# Autodesk Inventor assembly: _MK-1_Assembly
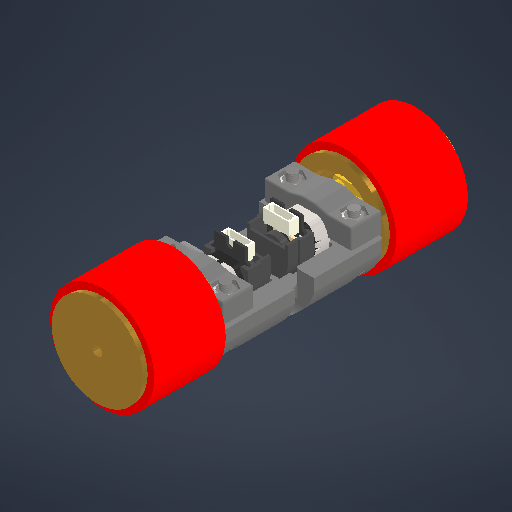
[picture p0: Inventor's stored thumbnail of the model, 512x512]
Saved by Autodesk Inventor 2027 (Build 310192000, 192)
## iProperties
Created: 2026-04-22
Part Number: _MK-1_Assembly
Document SubType Name: Assembly
Designer: Vadim
Author: Vadim
## Documents named in this file (12)
- C:\Users\Vadim\GitHub\NeoSumec\NeoSumec-MiniSumo-MECH\_MK-1_\_MK-1_Assembly.iam
- C:\Users\Vadim\GitHub\NeoSumec\NeoSumec-MiniSumo-MECH\_MK-1_\Models\3D_Print\MotorMountBottom.ipt
- C:\Users\Vadim\GitHub\NeoSumec\NeoSumec-MiniSumo-MECH\_MK-1_\Models\3D_Print\MotorClamp.ipt
- C:\Users\Vadim\GitHub\NeoSumec\NeoSumec-MiniSumo-MECH\_MK-1_\Models\Metal\pipe.ipt
- C:\Users\Vadim\GitHub\NeoSumec\NeoSumec-MiniSumo-MECH\_MK-1_\Models\Metal\Wheel.ipt
- C:\Users\Vadim\GitHub\NeoSumec\NeoSumec-MiniSumo-MECH\_MK-1_\Models\3rd-party_comp\Pololu Micro Metal Gearmotor 3D (STEP) Models\With Encoder, Side Connector\mmgm-cb-enc-side-con\mmgm-cb-enc-side-con\mmgm-cb-enc-side-con.ipt
- C:\Users\Vadim\GitHub\NeoSumec\NeoSumec-MiniSumo-MECH\_MK-1_\Models\Other technology\silicon bublebum.ipt
- C:\Users\Vadim\GitHub\NeoSumec\NeoSumec-MiniSumo-MECH\_MK-1_\SpojMat\DIN 934 - M3 x 0,5.ipt
- C:\Users\Vadim\GitHub\NeoSumec\NeoSumec-MiniSumo-MECH\_MK-1_\SpojMat\ISO 14580 M3x25-4.8.ipt
- C:\Users\Vadim\GitHub\NeoSumec\NeoSumec-MiniSumo-MECH\_MK-1_\SpojMat\ISO 14581 - M3x16-4.8.ipt
- C:\Users\Vadim\GitHub\NeoSumec\NeoSumec-MiniSumo-MECH\_MK-1_\SpojMat\ISO 14581 - M3x20-4.8.ipt
- C:\Users\Vadim\GitHub\NeoSumec\NeoSumec-MiniSumo-MECH\_MK-1_\SpojMat\DIN 916 - M3  x  6.ipt
## Components (23 placed, 11 different names)
1. MotorMountBottom:1 — Proti sobě:1, Proti sobě:2, Proti sobě:3, Proti sobě:4, Proti sobě:7, Proti sobě:10, Proti sobě:15, Stejný směr:1, Proti sobě:17, Proti sobě:19, Proti sobě:21, Proti sobě:34, Proti sobě:35, Proti sobě:36, Proti sobě:37, Proti sobě:38, Proti sobě:39, Proti sobě:40, Proti sobě:41
2. MotorClamp:1 — Proti sobě:18, Proti sobě:19, Proti sobě:24, Proti sobě:25, Proti sobě:26, Proti sobě:27, Proti sobě:32, Proti sobě:33
3. MotorClamp:2 — Proti sobě:16, Proti sobě:17, Proti sobě:22, Proti sobě:23, Proti sobě:28, Proti sobě:29, Proti sobě:30, Proti sobě:31
4. pipe:1 — Proti sobě:15, Stejný směr:1, Proti sobě:20
5. Wheel:1 — Proti sobě:5, Proti sobě:6, Proti sobě:7, Proti sobě:11, Proti sobě:14, Proti sobě:42, Proti sobě:44
6. Wheel:2 — Proti sobě:8, Proti sobě:9, Proti sobě:10, Proti sobě:12, Proti sobě:13, Proti sobě:45, Proti sobě:46
7. silicon bublebum:1 — Proti sobě:11, Proti sobě:14
8. silicon bublebum:2 — Proti sobě:12, Proti sobě:13
9. mmgm-cb-enc-side-con:1 — Proti sobě:1, Proti sobě:2, Proti sobě:5, Proti sobě:6, Proti sobě:18, Proti sobě:43, Proti sobě:49
10. mmgm-cb-enc-side-con:2 — Proti sobě:3, Proti sobě:4, Proti sobě:8, Proti sobě:9, Proti sobě:16, Proti sobě:47, Proti sobě:48
11. ISO 14580 M3x25-4.8:1 — Proti sobě:20, Proti sobě:21
12. DIN 916 - M3  x  6:1 — Proti sobě:42, Proti sobě:43
13. DIN 916 - M3  x  6:2 — Proti sobě:44, Proti sobě:49
14. DIN 916 - M3  x  6:3 — Proti sobě:45, Proti sobě:47
15. DIN 916 - M3  x  6:4 — Proti sobě:46, Proti sobě:48
16. ISO 14581 - M3x16-4.8:1 — Proti sobě:36, Proti sobě:37
17. ISO 14581 - M3x16-4.8:2 — Proti sobě:38, Proti sobě:39
18. ISO 14581 - M3x20-4.8:1 — Proti sobě:34, Proti sobě:35
19. ISO 14581 - M3x20-4.8:2 — Proti sobě:40, Proti sobě:41
20. DIN 934 - M3 x 0,5:1 — Proti sobě:25, Proti sobě:26, Proti sobě:33
21. DIN 934 - M3 x 0,5:2 — Proti sobě:24, Proti sobě:27, Proti sobě:32
22. DIN 934 - M3 x 0,5:3 — Proti sobě:22, Proti sobě:29, Proti sobě:30
23. DIN 934 - M3 x 0,5:4 — Proti sobě:23, Proti sobě:28, Proti sobě:31
## Relationships (50: Mate 49, Flush 1)
- Proti sobě:1 [Mate]: MotorMountBottom:1 ↔ mmgm-cb-enc-side-con:1
- Proti sobě:2 [Mate] (0.125 mm): MotorMountBottom:1 ↔ mmgm-cb-enc-side-con:1
- Proti sobě:3 [Mate]: MotorMountBottom:1 ↔ mmgm-cb-enc-side-con:2
- Proti sobě:4 [Mate] (0.125 mm): MotorMountBottom:1 ↔ mmgm-cb-enc-side-con:2
- Proti sobě:5 [Mate]: Wheel:1 ↔ mmgm-cb-enc-side-con:1
- Proti sobě:6 [Mate] (0.1 mm): Wheel:1 ↔ mmgm-cb-enc-side-con:1
- Proti sobě:7 [Mate] (0.25 mm): MotorMountBottom:1 ↔ Wheel:1
- Proti sobě:8 [Mate]: Wheel:2 ↔ mmgm-cb-enc-side-con:2
- Proti sobě:9 [Mate] (0.15 mm): Wheel:2 ↔ mmgm-cb-enc-side-con:2
- Proti sobě:10 [Mate] (0.25 mm): MotorMountBottom:1 ↔ Wheel:2
- Proti sobě:11 [Mate]: Wheel:1 ↔ silicon bublebum:1
- Proti sobě:12 [Mate]: Wheel:2 ↔ silicon bublebum:2
- Proti sobě:13 [Mate]: Wheel:2 ↔ silicon bublebum:2
- Proti sobě:14 [Mate]: Wheel:1 ↔ silicon bublebum:1
- Proti sobě:15 [Mate]: MotorMountBottom:1 ↔ pipe:1
- Stejný směr:1 [Flush]: MotorMountBottom:1 ↔ pipe:1
- Proti sobě:16 [Mate]: MotorClamp:2 ↔ mmgm-cb-enc-side-con:2
- Proti sobě:17 [Mate]: MotorMountBottom:1 ↔ MotorClamp:2
- Proti sobě:18 [Mate]: MotorClamp:1 ↔ mmgm-cb-enc-side-con:1
- Proti sobě:19 [Mate]: MotorMountBottom:1 ↔ MotorClamp:1
- Proti sobě:20 [Mate]: pipe:1 ↔ ISO 14580 M3x25-4.8:1
- Proti sobě:21 [Mate]: MotorMountBottom:1 ↔ ISO 14580 M3x25-4.8:1
- Proti sobě:22 [Mate]: MotorClamp:2 ↔ DIN 934 - M3 x 0,5:3
- Proti sobě:23 [Mate]: MotorClamp:2 ↔ DIN 934 - M3 x 0,5:4
- Proti sobě:24 [Mate]: MotorClamp:1 ↔ DIN 934 - M3 x 0,5:2
- Proti sobě:25 [Mate]: MotorClamp:1 ↔ DIN 934 - M3 x 0,5:1
- Proti sobě:26 [Mate] (0.1 mm): MotorClamp:1 ↔ DIN 934 - M3 x 0,5:1
- Proti sobě:27 [Mate] (0.1 mm): MotorClamp:1 ↔ DIN 934 - M3 x 0,5:2
- Proti sobě:28 [Mate] (0.1 mm): MotorClamp:2 ↔ DIN 934 - M3 x 0,5:4
- Proti sobě:29 [Mate] (0.1 mm): MotorClamp:2 ↔ DIN 934 - M3 x 0,5:3
- Proti sobě:30 [Mate]: MotorClamp:2 ↔ DIN 934 - M3 x 0,5:3
- Proti sobě:31 [Mate]: MotorClamp:2 ↔ DIN 934 - M3 x 0,5:4
- Proti sobě:32 [Mate]: MotorClamp:1 ↔ DIN 934 - M3 x 0,5:2
- Proti sobě:33 [Mate]: MotorClamp:1 ↔ DIN 934 - M3 x 0,5:1
- Proti sobě:34 [Mate]: MotorMountBottom:1 ↔ ISO 14581 - M3x20-4.8:1
- Proti sobě:35 [Mate]: MotorMountBottom:1 ↔ ISO 14581 - M3x20-4.8:1
- Proti sobě:36 [Mate]: MotorMountBottom:1 ↔ ISO 14581 - M3x16-4.8:1
- Proti sobě:37 [Mate]: MotorMountBottom:1 ↔ ISO 14581 - M3x16-4.8:1
- Proti sobě:38 [Mate]: MotorMountBottom:1 ↔ ISO 14581 - M3x16-4.8:2
- Proti sobě:39 [Mate]: MotorMountBottom:1 ↔ ISO 14581 - M3x16-4.8:2
- Proti sobě:40 [Mate]: MotorMountBottom:1 ↔ ISO 14581 - M3x20-4.8:2
- Proti sobě:41 [Mate]: MotorMountBottom:1 ↔ ISO 14581 - M3x20-4.8:2
- Proti sobě:42 [Mate]: Wheel:1 ↔ DIN 916 - M3  x  6:1
- Proti sobě:43 [Mate]: mmgm-cb-enc-side-con:1 ↔ DIN 916 - M3  x  6:1
- Proti sobě:44 [Mate]: Wheel:1 ↔ DIN 916 - M3  x  6:2
- Proti sobě:45 [Mate]: Wheel:2 ↔ DIN 916 - M3  x  6:3
- Proti sobě:46 [Mate]: Wheel:2 ↔ DIN 916 - M3  x  6:4
- Proti sobě:47 [Mate]: mmgm-cb-enc-side-con:2 ↔ DIN 916 - M3  x  6:3
- Proti sobě:48 [Mate]: mmgm-cb-enc-side-con:2 ↔ DIN 916 - M3  x  6:4
- Proti sobě:49 [Mate]: mmgm-cb-enc-side-con:1 ↔ DIN 916 - M3  x  6:2
